# Autodesk Inventor assembly: butelka
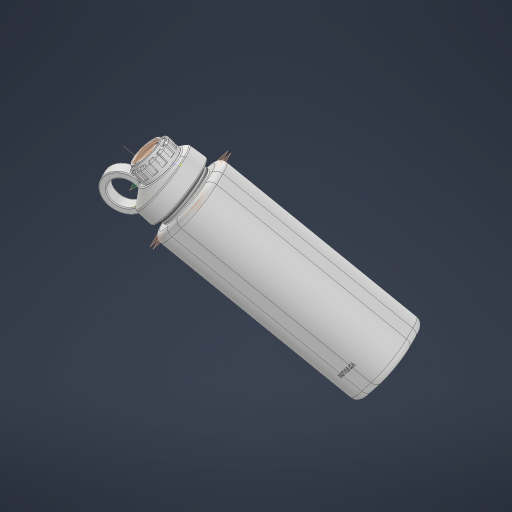
[picture p0: Inventor's stored thumbnail of the model, 512x512]
Saved by Autodesk Inventor 2023 (Build 270158000, 158)
## iProperties
Created: 2023-05-18
Part Number: butelka
Document SubType Name: Assembly
Designer: Adam
Author: Adam
## Documents named in this file (6)
- C:\Users\pryst\Desktop\KoNaR\Warsztaty\Mechanika\Projekty\Adam_Prystupa\BUTELKA\butelka.iam
- C:\Users\pryst\Desktop\KoNaR\Warsztaty\Mechanika\Projekty\Adam_Prystupa\BUTELKA\Część1.ipt
- C:\Users\pryst\Desktop\KoNaR\Warsztaty\Mechanika\Projekty\Adam_Prystupa\BUTELKA\Część2.ipt
- C:\Users\pryst\Desktop\KoNaR\Warsztaty\Mechanika\Projekty\Adam_Prystupa\BUTELKA\Część3.ipt
- C:\Users\pryst\Desktop\KoNaR\Warsztaty\Mechanika\Projekty\Adam_Prystupa\BUTELKA\Część4.ipt
- C:\Users\pryst\Desktop\KoNaR\Warsztaty\Mechanika\Projekty\Adam_Prystupa\BUTELKA\Część5.ipt
## Components (5 placed, 5 different names)
1. Część1:1 — Kątowe:1
2. Część2:1 — Kątowe:1, Kątowe:2, Przejściowe:1, Zestawiające:1
3. Część3:1 — Obrotowe:1
4. Część4:1 — Obrotowe:1, Obrotowe:2, Zestawiające:1
5. Część5:1 — Obrotowe:2, Kątowe:2, Przejściowe:1
## Relationships (6: Angle 2, RevoluteJoint 2, Transitional 1, Mate 1)
- Kątowe:1 [Angle] (0 deg): Część1:1 ↔ Część2:1
- Obrotowe:1 [RevoluteJoint] (3 mm): Część3:1 ↔ Część4:1
- Obrotowe:2 [RevoluteJoint]: Część4:1 ↔ Część5:1
- Kątowe:2 [Angle] (180 deg): Część2:1 ↔ Część5:1
- Przejściowe:1 [Transitional]: Część2:1 ↔ Część5:1
- Zestawiające:1 [Mate] (0.25 mm): Część2:1 ↔ Część4:1
